# Autodesk Inventor assembly: Gripper Assembly
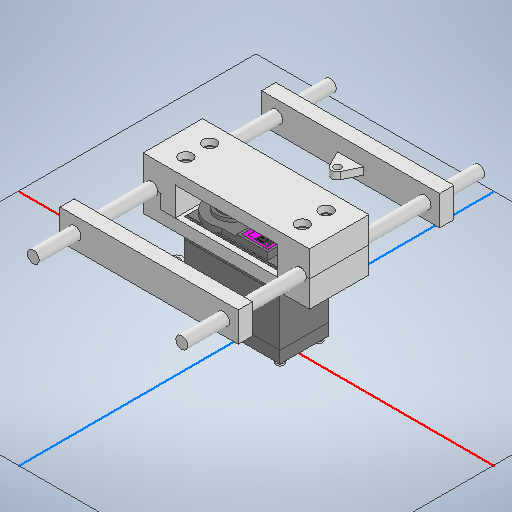
[picture p0: Inventor's stored thumbnail of the model, 512x512]
Saved by Autodesk Inventor 2025.2 (Build 292293000, 293)
## iProperties
Created: 2025-01-12
Part Number: Gripper Assembly
Document SubType Name: Assembly
Designer: caomi
Author: caomi
## Documents named in this file (6)
- C:\Minh Nguyen\H2A\cad\Gripper\Gripper Assembly.iam
- C:\Minh Nguyen\H2A\cad\Gripper\Servo mount.ipt
- C:\Minh Nguyen\H2A\cad\Gripper\Servo_mount_front.ipt
- C:\Minh Nguyen\H2A\cad\Gripper\Linear Rod.ipt
- C:\Minh Nguyen\H2A\cad\Gripper\mg996R_v2\mg996R_v2\mg996R_v2.ipt
- C:\Minh Nguyen\H2A\cad\Gripper\Gripper_arms.ipt
## Components (7 placed, 5 different names)
1. Servo mount:1 — Mate:1, Mate:2, Insert:3, Insert:4
2. Servo_mount_front:1 — Mate:1, Mate:2, Insert:1, Insert:2
3. Linear Rod:1 — Insert:1, Cylindrical:1, Cylindrical:3
4. Linear Rod:2 — Insert:2, Cylindrical:2, Cylindrical:4
5. mg996R_v2:1 — Insert:3, Insert:4
6. Gripper_arms:1 — Cylindrical:1, Cylindrical:2
7. Gripper_arms:2 — Cylindrical:3, Cylindrical:4
## Relationships (10: Insert 4, CylindricalJoint 4, Mate 2)
- Mate:1: Servo mount:1 ↔ Servo_mount_front:1
- Mate:2: Servo mount:1 ↔ Servo_mount_front:1
- Insert:1: Servo_mount_front:1 ↔ Linear Rod:1
- Insert:2: Servo_mount_front:1 ↔ Linear Rod:2
- Insert:3: Servo mount:1 ↔ mg996R_v2:1
- Insert:4: Servo mount:1 ↔ mg996R_v2:1
- Cylindrical:1: Linear Rod:1 ↔ Gripper_arms:1
- Cylindrical:2: Linear Rod:2 ↔ Gripper_arms:1
- Cylindrical:3: Linear Rod:1 ↔ Gripper_arms:2
- Cylindrical:4: Linear Rod:2 ↔ Gripper_arms:2
